# Autodesk Inventor assembly: правая лапа - сборка
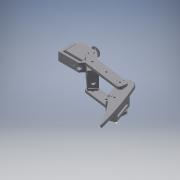
[picture p0: Inventor's stored thumbnail of the model, 180x180]
Saved by Autodesk Inventor 2019 (Build 230136000, 136)
## iProperties
Created: 2019-09-07
Part Number: правая лапа - сборка
Material: Типовые
Document SubType Name: Assembly
Designer: Iliga
Author: Iliga
## Documents named in this file (7)
- C:\Users\Iliga\Desktop\робот\правая лапа - сборка.iam
- C:\Users\Iliga\Desktop\робот\Юля\kreplenie4.ipt
- C:\Users\Iliga\Desktop\робот\двигатель.ipt
- C:\Users\Iliga\Desktop\робот\Юля\kreplenie1.ipt
- C:\Users\Iliga\Desktop\робот\Юля\peregorodka.ipt
- C:\Users\Iliga\Desktop\робот\Юля\kreplenie2.ipt
- C:\Users\Iliga\Desktop\робот\Юля\ship.ipt
## Components (9 placed, 6 different names)
1. kreplenie4:1 — Совмещение:1, Совмещение:2, Совмещение:3, Совмещение:4, Совмещение:5, Совмещение:6
2. двигатель:1 — Совмещение:1, Совмещение:2, Совмещение:3
3. двигатель:2 — Совмещение:7, Совмещение:8, Совмещение:9, Совмещение:10, Совмещение:11
4. двигатель:3 — Совмещение:16, Совмещение:18, Совмещение:19, Совмещение:20, Совмещение:21, Совмещение:22, Совмещение:23
5. kreplenie1:1 — Совмещение:4, Совмещение:5, Совмещение:6, Совмещение:7, Совмещение:8, Совмещение:9, Совмещение:12, Совмещение:13
6. peregorodka:1 — Совмещение:10, Совмещение:11, Совмещение:15, Совмещение:17
7. peregorodka:2 — Совмещение:12, Совмещение:13, Совмещение:20
8. kreplenie2:1 — Совмещение:15, Совмещение:16, Совмещение:17, Совмещение:18, Совмещение:19
9. ship:1 — Совмещение:21, Совмещение:22, Совмещение:23
## Relationships (22: Mate 22)
- Совмещение:1 [Mate]: kreplenie4:1 ↔ двигатель:1
- Совмещение:2 [Mate]: kreplenie4:1 ↔ двигатель:1
- Совмещение:3 [Mate]: kreplenie4:1 ↔ двигатель:1
- Совмещение:4 [Mate]: kreplenie4:1 ↔ kreplenie1:1
- Совмещение:5 [Mate]: kreplenie4:1 ↔ kreplenie1:1
- Совмещение:6 [Mate]: kreplenie4:1 ↔ kreplenie1:1
- Совмещение:7 [Mate]: двигатель:2 ↔ kreplenie1:1
- Совмещение:8 [Mate]: двигатель:2 ↔ kreplenie1:1
- Совмещение:9 [Mate]: двигатель:2 ↔ kreplenie1:1
- Совмещение:10 [Mate]: двигатель:2 ↔ peregorodka:1
- Совмещение:11 [Mate]: двигатель:2 ↔ peregorodka:1
- Совмещение:12 [Mate]: kreplenie1:1 ↔ peregorodka:2
- Совмещение:13 [Mate]: kreplenie1:1 ↔ peregorodka:2
- Совмещение:15 [Mate]: peregorodka:1 ↔ kreplenie2:1
- Совмещение:16 [Mate]: двигатель:3 ↔ kreplenie2:1
- Совмещение:17 [Mate]: peregorodka:1 ↔ kreplenie2:1
- Совмещение:18 [Mate]: двигатель:3 ↔ kreplenie2:1
- Совмещение:19 [Mate]: двигатель:3 ↔ kreplenie2:1
- Совмещение:20 [Mate]: двигатель:3 ↔ peregorodka:2
- Совмещение:21 [Mate]: двигатель:3 ↔ ship:1
- Совмещение:22 [Mate]: двигатель:3 ↔ ship:1
- Совмещение:23 [Mate]: двигатель:3 ↔ ship:1
